# Autodesk Inventor assembly: 吊架-短(R)(#01.05) - 焊接組合_MIR
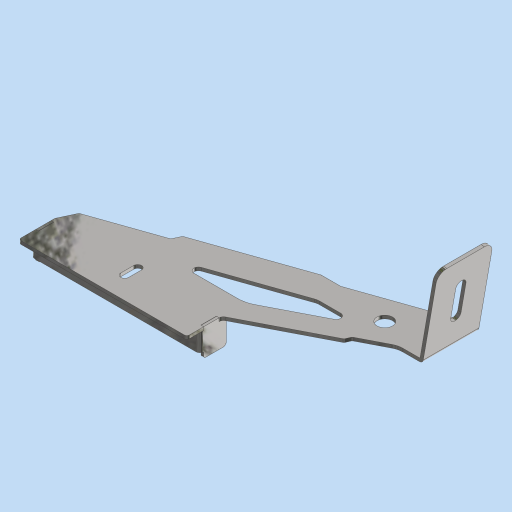
[picture p0: Inventor's stored thumbnail of the model, 512x512]
Saved by Autodesk Inventor 2023 (Build 270158000, 158)
## iProperties
Created: 2015-11-28
Part Number: 吊架-短(R)(#01.05) - 焊接組合_MIR
Document SubType Name: Assembly
Designer: 德國牧羊犬
Author: 設計製圖
## Documents named in this file (3)
- D:\資料庫\設計-工業3D\【May club 】\得利卡-車頂燈架\模型、圖面\成品版本\短-車頂燈架-組合(v220714)\吊架-短(R) - 焊接組合_MIR(v220714).iam
- D:\資料庫\設計-工業3D\【May club 】\得利卡-車頂燈架\模型、圖面\成品版本\短-車頂燈架-組合(v220714)\吊架-短(R) - 焊接件-1(v220714)_MIR.ipt
- D:\資料庫\設計-工業3D\【May club 】\得利卡-車頂燈架\模型、圖面\成品版本\短-車頂燈架-組合(v220714)\吊架-短-焊接件-2(v220714)_MIR.ipt
## Components (2 placed, 2 different names)
1. 吊架-短(R) - 焊接件-1(v220714)_MIR:1 — 貼合:3, 貼合:2, 貼合:1
2. 吊架-短-焊接件-2(v220714)_MIR:1 — 貼合:3, 貼合:2, 貼合:1
## Relationships (3: Mate 2, Flush 1)
- 貼合:3 [Mate]: 吊架-短(R) - 焊接件-1(v220714)_MIR:1 ↔ 吊架-短-焊接件-2(v220714)_MIR:1
- 貼合:2 [Flush]: 吊架-短(R) - 焊接件-1(v220714)_MIR:1 ↔ 吊架-短-焊接件-2(v220714)_MIR:1
- 貼合:1 [Mate]: 吊架-短(R) - 焊接件-1(v220714)_MIR:1 ↔ 吊架-短-焊接件-2(v220714)_MIR:1
